# Autodesk Inventor assembly: project mikro
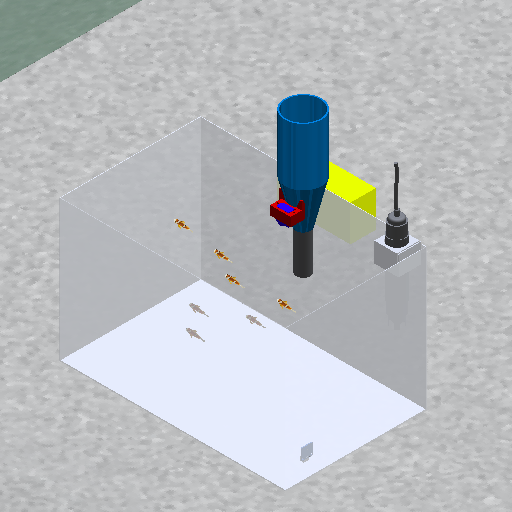
[picture p0: Inventor's stored thumbnail of the model, 512x512]
Saved by Autodesk Inventor 2027 (Build 310192060, 192F)
## iProperties
Created: 2026-06-09
Part Number: project mikro
Document SubType Name: Assembly
Designer: ridho
Author: ridho
## Documents named in this file (13)
- C:\Users\ridho\OneDrive\Dokumen\project mikro.iam
- C:\Users\ridho\Downloads\rtc-module-ds3231-1.snapshot.1\DS3231-module\DS3231-module.ipt
- C:\Users\ridho\OneDrive\Dokumen\aquariuu.ipt
- C:\Users\ridho\OneDrive\Dokumen\Box .ipt
- C:\Users\ridho\OneDrive\Dokumen\Part16.ipt
- C:\Users\ridho\OneDrive\Dokumen\Part6.ipt
- C:\Users\ridho\OneDrive\Dokumen\pipa.ipt
- C:\Users\ridho\Downloads\arduino-mega-17.snapshot.19\Arduino Mega 2560\Arduino Mega 2560.ipt
- C:\Users\ridho\Downloads\ph-sensor-1.snapshot.1\pH_Sensor\pH_Sensor.ipt
- C:\Users\ridho\Downloads\sg90-servo-motor-6.snapshot.6\SG-90_Motor\SG-90_Motor.ipt
- C:\Users\ridho\Downloads\sunfounder-ds18b20-1.snapshot.11\SunFounder DS18B20 v3\SunFounder DS18B20 v3.ipt
- C:\Users\ridho\OneDrive\Dokumen\Bracket PH.ipt
- C:\Users\ridho\Downloads\sunfounder-ds18b20-1.snapshot.11\12265_Fish_v1_L2.ipt
## Components (18 placed, 12 different names)
1. DS3231-module:1 — Rigid:3
2. aquariuu:1 — Rigid:1, Rigid:2, Mate:1, Mate:2
3. Box :1 — Rigid:2, Rotational:2, Rigid:3
4. Part16:1 — Rotational:1, Cylindrical:1, Rigid:1
5. Part6:1 — Insert:1
6. pipa:1 — Insert:1, Cylindrical:1
7. Arduino Mega 2560:1 — Rotational:2
8. SG-90_Motor:1 — Rotational:1
9. Bracket PH:1 — Rigid:4, Mate:1
10. pH_Sensor:1 — Rigid:4
11. SunFounder DS18B20 v3:1 — Mate:2
12. 12265_Fish_v1_L2:1
13. 12265_Fish_v1_L2:2
14. 12265_Fish_v1_L2:3
15. 12265_Fish_v1_L2:4
16. 12265_Fish_v1_L2:5
17. 12265_Fish_v1_L2:6
18. 12265_Fish_v1_L2:7
## Relationships (10: WeldJoint 4, RevoluteJoint 2, Mate 2, Insert 1, CylindricalJoint 1)
- Insert:1: Part6:1 ↔ pipa:1
- Rotational:1 [RevoluteJoint]: Part16:1 ↔ SG-90_Motor:1
- Cylindrical:1: Part16:1 ↔ pipa:1
- Rigid:1 [WeldJoint]: aquariuu:1 ↔ Part16:1
- Rigid:2 [WeldJoint]: aquariuu:1 ↔ Box :1
- Rotational:2 [RevoluteJoint]: Box :1 ↔ Arduino Mega 2560:1
- Rigid:3 [WeldJoint]: DS3231-module:1 ↔ Box :1
- Rigid:4 [WeldJoint] (-120 mm): Bracket PH:1 ↔ pH_Sensor:1
- Mate:1: aquariuu:1 ↔ Bracket PH:1
- Mate:2: aquariuu:1 ↔ SunFounder DS18B20 v3:1
